# Autodesk Inventor assembly: switchplate-2
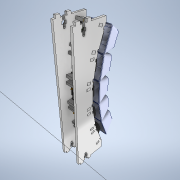
[picture p0: Inventor's stored thumbnail of the model, 180x180]
Saved by Autodesk Inventor 2020 (Build 240168000, 168)
## iProperties
Created: 2019-07-06
Part Number: switchplate-2
Document SubType Name: Assembly
Designer: Thibault
Mass: 36.7321 g
Surface Area: 336.688 cm^2
Volume: 13.7102 cm^3
Density: 2.67918 g/cm^3
Author: Thibault
## Documents named in this file (7)
- C:\Users\Thibault Polge\Documents\Habilis\mech\switchplate\switchplate-2.iam
- C:\Users\Thibault Polge\Documents\Habilis\mech\switchplate_support.ipt
- C:\Users\Thibault Polge\Documents\Habilis\mech\mx.iam
- C:\Users\Thibault Polge\Documents\Habilis\mech\extra_switch_support.ipt
- C:\Users\Thibault Polge\Documents\Habilis\mech\mx\SA-R3.iam
- C:\Users\Thibault Polge\Documents\Habilis\mech\switchplate.iam
- C:\Users\Thibault Polge\Documents\Habilis\mech\switchplate_support\switchplate-support-02.ipt
## Components (17 placed, 4 different names)
1. switchplate-support:left — Affleurement:1, Affleurement:2, Affleurement:3, Affleurement:5, Placage:1, Placage:2, Placage:3, Placage:4, Placage:5, Placage:6, Placage:7, Placage:8, Placage:9, Placage:10, Affleurement:6, Affleurement:7, Affleurement:8, Affleurement:9, Affleurement:10, Affleurement:11, Affleurement:12, Affleurement:13, Affleurement:14, Affleurement:15, Placage:11, Placage:12, Placage:13, Placage:14, Placage:15, Placage:16, Placage:17, Placage:18, Placage:19, Placage:20, Affleurement:17, Symétrie:1
2. Switch:1 [sub-assembly] — Placage:26, Affleurement:22, Placage:35
3. Switch:2 [sub-assembly] — Placage:30, Affleurement:21, Placage:34
4. Switch:3 [sub-assembly] — Placage:27, Affleurement:20, Placage:33
5. Switch:4 [sub-assembly] — Placage:28, Affleurement:19, Placage:32
6. Switch:5 [sub-assembly] — Placage:29, Affleurement:18, Placage:31
7. switchplate-support:right — Affleurement:5, Affleurement:16, Affleurement:17, Symétrie:1
8. extra_switch_support:1 — Placage:1, Affleurement:13, Placage:18, Placage:30
9. extra_switch_support:2 — Placage:2, Affleurement:12, Placage:17, Placage:34
10. extra_switch_support:3 — Placage:3, Affleurement:11, Placage:16, Placage:27
11. extra_switch_support:4 — Placage:4, Affleurement:10, Placage:15, Placage:33
12. extra_switch_support:5 — Placage:5, Affleurement:9, Placage:14, Placage:28
13. extra_switch_support:6 — Placage:6, Affleurement:8, Placage:13, Placage:32
14. extra_switch_support:7 — Placage:7, Affleurement:7, Placage:12, Placage:29
15. extra_switch_support:8 — Placage:9, Affleurement:14, Placage:19, Placage:35
16. extra_switch_support:9 — Placage:10, Affleurement:15, Placage:20, Placage:26
17. extra_switch_support:10 — Placage:8, Affleurement:6, Placage:11, Affleurement:16, Placage:31
## Relationships (52: Mate 30, Flush 21, Symmetry 1)
- Affleurement:1 [Flush]: switchplate-support:left
- Affleurement:2 [Flush]: switchplate-support:left
- Affleurement:3 [Flush]: switchplate-support:left
- Affleurement:5 [Flush]: switchplate-support:left ↔ switchplate-support:right
- Placage:1 [Mate]: switchplate-support:left ↔ extra_switch_support:1
- Placage:2 [Mate]: switchplate-support:left ↔ extra_switch_support:2
- Placage:3 [Mate]: switchplate-support:left ↔ extra_switch_support:3
- Placage:4 [Mate]: switchplate-support:left ↔ extra_switch_support:4
- Placage:5 [Mate]: switchplate-support:left ↔ extra_switch_support:5
- Placage:6 [Mate]: switchplate-support:left ↔ extra_switch_support:6
- Placage:7 [Mate]: switchplate-support:left ↔ extra_switch_support:7
- Placage:8 [Mate]: switchplate-support:left ↔ extra_switch_support:10
- Placage:9 [Mate]: switchplate-support:left ↔ extra_switch_support:8
- Placage:10 [Mate]: switchplate-support:left ↔ extra_switch_support:9
- Affleurement:6 [Flush]: switchplate-support:left ↔ extra_switch_support:10
- Affleurement:7 [Flush]: switchplate-support:left ↔ extra_switch_support:7
- Affleurement:8 [Flush]: switchplate-support:left ↔ extra_switch_support:6
- Affleurement:9 [Flush]: switchplate-support:left ↔ extra_switch_support:5
- Affleurement:10 [Flush]: switchplate-support:left ↔ extra_switch_support:4
- Affleurement:11 [Flush]: switchplate-support:left ↔ extra_switch_support:3
- Affleurement:12 [Flush]: switchplate-support:left ↔ extra_switch_support:2
- Affleurement:13 [Flush]: switchplate-support:left ↔ extra_switch_support:1
- Affleurement:14 [Flush]: switchplate-support:left ↔ extra_switch_support:8
- Affleurement:15 [Flush]: switchplate-support:left ↔ extra_switch_support:9
- Placage:11 [Mate]: switchplate-support:left ↔ extra_switch_support:10
- Placage:12 [Mate]: switchplate-support:left ↔ extra_switch_support:7
- Placage:13 [Mate]: switchplate-support:left ↔ extra_switch_support:6
- Placage:14 [Mate]: switchplate-support:left ↔ extra_switch_support:5
- Placage:15 [Mate]: switchplate-support:left ↔ extra_switch_support:4
- Placage:16 [Mate]: switchplate-support:left ↔ extra_switch_support:3
- Placage:17 [Mate]: switchplate-support:left ↔ extra_switch_support:2
- Placage:18 [Mate]: switchplate-support:left ↔ extra_switch_support:1
- Placage:19 [Mate]: switchplate-support:left ↔ extra_switch_support:8
- Placage:20 [Mate]: switchplate-support:left ↔ extra_switch_support:9
- Affleurement:16 [Flush]: switchplate-support:right ↔ extra_switch_support:10
- Affleurement:17 [Flush]: switchplate-support:left ↔ switchplate-support:right
- Symétrie:1 [Symmetry]: switchplate-support:left ↔ switchplate-support:right
- Placage:26 [Mate]: Switch:1 ↔ extra_switch_support:9
- Placage:27 [Mate]: Switch:3 ↔ extra_switch_support:3
- Placage:28 [Mate]: Switch:4 ↔ extra_switch_support:5
- Placage:29 [Mate]: Switch:5 ↔ extra_switch_support:7
- Placage:30 [Mate]: Switch:2 ↔ extra_switch_support:1
- Affleurement:18 [Flush]: Switch:5
- Affleurement:19 [Flush]: Switch:4
- Affleurement:20 [Flush]: Switch:3
- Affleurement:21 [Flush]: Switch:2
- Affleurement:22 [Flush]: Switch:1
- Placage:31 [Mate]: Switch:5 ↔ extra_switch_support:10
- Placage:32 [Mate]: Switch:4 ↔ extra_switch_support:6
- Placage:33 [Mate]: Switch:3 ↔ extra_switch_support:4
- Placage:34 [Mate]: Switch:2 ↔ extra_switch_support:2
- Placage:35 [Mate]: Switch:1 ↔ extra_switch_support:8
